# Autodesk Inventor assembly: sensorHolder
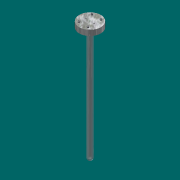
[picture p0: Inventor's stored thumbnail of the model, 180x180]
Saved by Autodesk Inventor 2016 (Build 200138000, 138)
## iProperties
Created: 2016-09-24
Part Number: sensorHolder
Document SubType Name: Assembly
Designer: sawaiz
Author: sawaiz
## Documents named in this file (6)
- C:\Users\sawaiz\oneDrive\projects\neutronCell\sensorHolder.iam
- C:\Users\sawaiz\oneDrive\projects\neutronCell\sensorHolder.ipt
- C:\Users\sawaiz\oneDrive\projects\neutronCell\glassTube.ipt
- C:\Users\sawaiz\oneDrive\projects\neutronCell\fiber.ipt
- C:\Users\sawaiz\oneDrive\projects\neutronCell\oRing.ipt
- C:\Users\sawaiz\oneDrive\projects\neutronCell\4-40SocketCap0.625.ipt
## Components (8 placed, 5 different names)
1. sensorHolder:1 — Mate:1, Flush:1, Mate:2, Mate:3, Mate:4, Mate:5, Mate:6, Mate:7, Mate:8, Mate:9, Mate:10
2. glassTube:1 — Mate:2, Mate:3
3. fiber:1 — Mate:1, Flush:1
4. oRing:1 — Mate:4, Mate:5
5. 4-40SocketCap0.625:1 — Flush:2, Mate:6, Mate:8
6. 4-40SocketCap0.625:2 — Flush:2, Flush:4, Mate:9
7. 4-40SocketCap0.625:3 — Flush:3, Flush:4, Mate:10
8. 4-40SocketCap0.625:4 — Flush:3, Mate:7
## Relationships (14: Mate 10, Flush 4)
- Mate:1: sensorHolder:1 ↔ fiber:1
- Flush:1 (-1 mm): sensorHolder:1 ↔ fiber:1
- Mate:2: sensorHolder:1 ↔ glassTube:1
- Mate:3: sensorHolder:1 ↔ glassTube:1
- Mate:4: sensorHolder:1 ↔ oRing:1
- Mate:5: sensorHolder:1 ↔ oRing:1
- Flush:2: 4-40SocketCap0.625:1 ↔ 4-40SocketCap0.625:2
- Flush:3: 4-40SocketCap0.625:3 ↔ 4-40SocketCap0.625:4
- Flush:4: 4-40SocketCap0.625:2 ↔ 4-40SocketCap0.625:3
- Mate:6: sensorHolder:1 ↔ 4-40SocketCap0.625:1
- Mate:7: sensorHolder:1 ↔ 4-40SocketCap0.625:4
- Mate:8: sensorHolder:1 ↔ 4-40SocketCap0.625:1
- Mate:9: sensorHolder:1 ↔ 4-40SocketCap0.625:2
- Mate:10: sensorHolder:1 ↔ 4-40SocketCap0.625:3
